# Autodesk Inventor assembly: RearWheelNoLogo
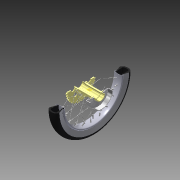
[picture p0: Inventor's stored thumbnail of the model, 180x180]
Saved by Autodesk Inventor 2016 (Build 200138000, 138)
## iProperties
Shininess: 20.0
Length Units: 11272
Angle Units: 11279
Time Units: 11290
Mass Units: 11286
Length Display Precision: 3
Angle Display Precision: 2
Compacted: True
Created: 2001-05-25
Part Number: RearWheelNoLogo
Document SubType Name: Assembly
Designer: Administrator
Density: 0.0
Volumn: 0.0
Area: 0.0
PropertySet Name: Model Information
Control State: 0
Master: False
Checked Out: False
Author: Administrator
## Documents named in this file (8)
- C:\Users\Yann\Documents\GitHub\BIKAIR_CAD\Source\Front_Train\Wheel_spokes\Wheel_spokes.iam
- C:\Users\Yann\Documents\GitHub\BIKAIR_CAD\Source\Front_Train\Wheel_spokes\RearHub.ipt
- C:\Users\Yann\Documents\GitHub\BIKAIR_CAD\Source\Front_Train\Wheel_spokes\ClincherRim2.ipt
- C:\Users\Yann\Documents\GitHub\BIKAIR_CAD\Source\Front_Train\Wheel_spokes\SpokeRear.ipt
- C:\Users\Yann\Documents\GitHub\BIKAIR_CAD\Source\Front_Train\Wheel_spokes\FrontTire.ipt
- C:\Users\Yann\Documents\GitHub\BIKAIR_CAD\Source\Front_Train\Wheel_spokes\RearSprocket.ipt
- C:\Users\Yann\Documents\GitHub\BIKAIR_CAD\Source\Front_Train\Wheel_spokes\BrakeDrum.ipt
- C:\Users\Yann\Documents\GitHub\BIKAIR_CAD\Source\Front_Train\Wheel_spokes\wheel_tyre.ipt
## Components (46 placed, 7 different names)
1. RearHub:1 — Mate:1, Mate:2, Mate:3, Mate:5, Mate:7, Mate:9, Mate:11, Insert:1, Insert:2
2. ClincherRim2:1 — Mate:1, Mate:3, Mate:4, Mate:6, Mate:8, Mate:10, Mate:12
3. FrontTire:1 — Mate:11, Mate:12
4. RearSprocket:1 — Insert:1
5. BrakeDrum:1 — Insert:2
6. wheel_tyre:1 — Mate:13, Mate:14
7. SpokeRear:1 — Mate:2, Mate:4
8. SpokeRear:2 — Mate:5, Mate:6
9. SpokeRear:3 — Mate:7, Mate:8
10. SpokeRear:4 — Mate:9, Mate:10
11. SpokeRear:5
12. SpokeRear:6
13. SpokeRear:7
14. SpokeRear:8
15. SpokeRear:9
16. SpokeRear:10
17. SpokeRear:11
18. SpokeRear:12
19. SpokeRear:13
20. SpokeRear:14
21. SpokeRear:15
22. SpokeRear:16
23. SpokeRear:17
24. SpokeRear:18
25. SpokeRear:19
26. SpokeRear:20
27. SpokeRear:21
28. SpokeRear:22
29. SpokeRear:23
30. SpokeRear:24
31. SpokeRear:25
32. SpokeRear:26
33. SpokeRear:27
34. SpokeRear:28
35. SpokeRear:29
36. SpokeRear:30
37. SpokeRear:31
38. SpokeRear:32
39. SpokeRear:33
40. SpokeRear:34
41. SpokeRear:35
42. SpokeRear:36
43. SpokeRear:37
44. SpokeRear:38
45. SpokeRear:39
46. SpokeRear:40
## Component patterns: (10 elements, first: SpokeRear:1 + SpokeRear:2 + SpokeRear:3 + SpokeRear:4)
## Relationships (16: Mate 14, Insert 2)
- Mate:1: RearHub:1 ↔ ClincherRim2:1
- Mate:2: RearHub:1 ↔ SpokeRear:1
- Mate:3: RearHub:1 ↔ ClincherRim2:1
- Mate:4: ClincherRim2:1 ↔ SpokeRear:1
- Mate:5: RearHub:1 ↔ SpokeRear:2
- Mate:6: ClincherRim2:1 ↔ SpokeRear:2
- Mate:7: RearHub:1 ↔ SpokeRear:3
- Mate:8: ClincherRim2:1 ↔ SpokeRear:3
- Mate:9: RearHub:1 ↔ SpokeRear:4
- Mate:10: ClincherRim2:1 ↔ SpokeRear:4
- Mate:11: RearHub:1 ↔ FrontTire:1
- Mate:12: ClincherRim2:1 ↔ FrontTire:1
- Insert:1: RearHub:1 ↔ RearSprocket:1
- Insert:2: RearHub:1 ↔ BrakeDrum:1
- Mate:13: wheel_tyre:1
- Mate:14: wheel_tyre:1
